# Autodesk Inventor assembly: chessboard-base
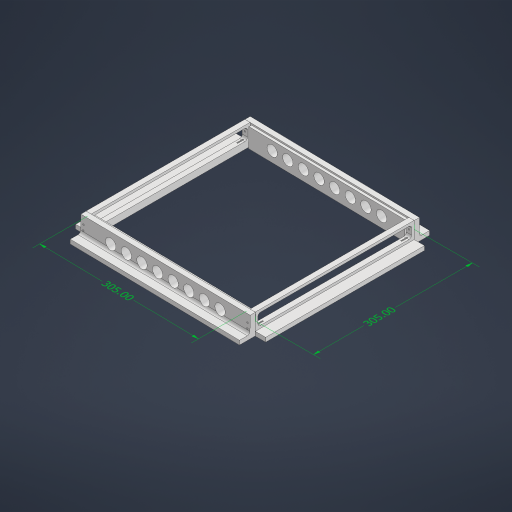
[picture p0: Inventor's stored thumbnail of the model, 512x512]
Saved by Autodesk Inventor 2023 (Build 270158000, 158)
## iProperties
Created: 2023-12-20
Part Number: chessboard-base
Document SubType Name: Assembly
Designer: hrush
Author: hrush
## Documents named in this file (3)
- C:\CAD\Robotic Arm 3D Model step\chessboard-base.iam
- C:\CAD\Robotic Arm 3D Model step\chessboard-base-1.ipt
- C:\CAD\Robotic Arm 3D Model step\chessboard-base-2.ipt
## Components (4 placed, 2 different names)
1. chessboard-base-1:1 — Mate:1, Mate:2, Mate:5, Mate:6
2. chessboard-base-1:2 — Mate:3, Mate:4, Mate:7
3. chessboard-base-2:1 — Mate:5, Mate:6, Mate:7
4. chessboard-base-2:2 — Mate:1, Mate:2, Mate:3, Mate:4
## Relationships (7: Mate 7)
- Mate:1: chessboard-base-1:1 ↔ chessboard-base-2:2
- Mate:2: chessboard-base-1:1 ↔ chessboard-base-2:2
- Mate:3: chessboard-base-1:2 ↔ chessboard-base-2:2
- Mate:4: chessboard-base-1:2 ↔ chessboard-base-2:2
- Mate:5: chessboard-base-1:1 ↔ chessboard-base-2:1
- Mate:6: chessboard-base-1:1 ↔ chessboard-base-2:1
- Mate:7: chessboard-base-1:2 ↔ chessboard-base-2:1
